# Autodesk Inventor assembly: Assembly1
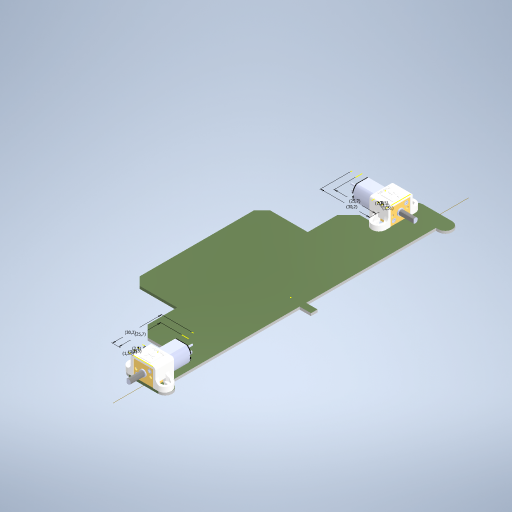
[picture p0: Inventor's stored thumbnail of the model, 512x512]
Saved by Autodesk Inventor 2024 (Build 280153000, 153)
## iProperties
Created: 2024-02-25
Part Number: Assembly1
Document SubType Name: Assembly
Designer: kamil
Author: kamil
## Documents named in this file (3)
- D:\Projects\Robotics\Hexapod\3DPrinterFiles\Assembly1.iam
- D:\Projects\Robotics\MaxVoltstapenV2\linefollower_chassy_model (1).ipt
- D:\Projects\Robotics\MaxVoltstapenV2\micro-metal-gearmotor-extended-with-1086-bracket\micro-metal-gearmotor-extended-with-1086-bracket.ipt
## Components (3 placed, 2 different names)
1. linefollower_chassy_model (1):1 — Mate:1, Mate:2
2. micro-metal-gearmotor-extended-with-1086-bracket:1
3. micro-metal-gearmotor-extended-with-1086-bracket:2 — Mate:1, Mate:2
## Relationships (2: Mate 2)
- Mate:1: linefollower_chassy_model (1):1 ↔ micro-metal-gearmotor-extended-with-1086-bracket:2
- Mate:2: linefollower_chassy_model (1):1 ↔ micro-metal-gearmotor-extended-with-1086-bracket:2
